# Autodesk Inventor assembly: case_assembly
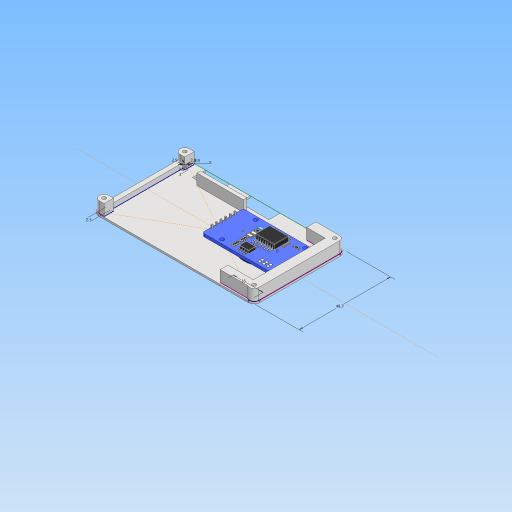
[picture p0: Inventor's stored thumbnail of the model, 512x512]
Saved by Autodesk Inventor 2023 (Build 270158000, 158)
## iProperties
Created: 2023-04-16
Part Number: case_assembly
Document SubType Name: Assembly
Designer: kar
Author: kar
## Documents named in this file (3)
- C:\Users\kar\Documents\Inventor\badgercase\case_assembly.iam
- C:\Users\kar\Documents\Inventor\badgercase\HW-84 v7.ipt
- C:\Users\kar\Documents\Inventor\badgercase\my_back_metric.ipt
## Components (2 placed, 2 different names)
1. HW-84 v7:1 — Mate:1, Angle:1, Mate:2, Mate:3
2. my_back_metric:1 — Mate:1, Angle:1, Mate:2, Mate:3
## Relationships (4: Mate 3, Angle 1)
- Mate:1 (0.762 mm): HW-84 v7:1 ↔ my_back_metric:1
- Angle:1 (180 deg): HW-84 v7:1 ↔ my_back_metric:1
- Mate:2: HW-84 v7:1 ↔ my_back_metric:1
- Mate:3: HW-84 v7:1 ↔ my_back_metric:1
